# Autodesk Inventor assembly: Gantry
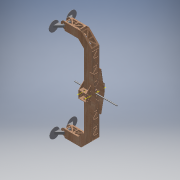
[picture p0: Inventor's stored thumbnail of the model, 180x180]
Saved by Autodesk Inventor 2019 (Build 230136000, 136)
## iProperties
Created: 2019-01-14
Part Number: Gantry
Document SubType Name: Assembly
Designer: nxgam
Author: nxgam
## Documents named in this file (8)
- C:\Users\nxgam\Documents\CAD\Inventor\DiscoDraw\Gantry.iam
- C:\Users\nxgam\Documents\CAD\Inventor\DiscoDraw\Shaft d10.ipt
- C:\Users\nxgam\Documents\CAD\Inventor\DiscoDraw\OctBase.ipt
- C:\Users\nxgam\Documents\CAD\Inventor\DiscoDraw\Leg.iam
- C:\Users\nxgam\Documents\CAD\Inventor\DiscoDraw\OctMiniSupport.ipt
- C:\Users\nxgam\Documents\CAD\Inventor\DiscoDraw\Flange.ipt
- C:\Users\nxgam\Documents\CAD\Inventor\DiscoDraw\SlipRing.ipt
- C:\Users\nxgam\Documents\CAD\Inventor\DiscoDraw\TrusSupport.ipt
## Components (14 placed, 7 different names)
1. Shaft d10:1 — Mate:3, Mate:11, Mate:14
2. OctBase:1 — Mate:1, Flush:3, Flush:4, Mate:2, Mate:3, Flush:14, Flush:15, Mate:13, Flush:16, Flush:19
3. OctBase:2 — Flush:3, Flush:4, Flush:6, Mate:4, Mate:5, Mate:6, Mate:7, Mate:12
4. Leg:1 [sub-assembly] — Flush:1, Flush:2, Mate:1, Flush:6, Flush:7, Angle:1, Flush:16, Mate:18
5. Leg:2 [sub-assembly] — Flush:1, Flush:2, Flush:7, Mate:2, Mate:16, Mate:17
6. OctMiniSupport:1 — Flush:11, Flush:12, Flush:15, Mate:6
7. OctMiniSupport:2 — Flush:10, Flush:11, Flush:12, Mate:7
8. OctMiniSupport:3 — Flush:9, Flush:10, Flush:13, Flush:14, Mate:5
9. OctMiniSupport:4 — Flush:9, Flush:13, Mate:4, Angle:3
10. Flange:1 — Mate:8, Angle:2, Mate:11, Mate:13
11. Flange:2 — Mate:8, Mate:12
12. SlipRing:1 — Mate:14, Angle:3
13. TrusSupport:1 — Mate:16, Flush:19, Flush:20, Flush:21
14. TrusSupport:2 — Mate:17, Flush:20, Flush:21, Mate:18
## Relationships (35: Flush 17, Mate 15, Angle 3)
- Flush:1: Leg:1 ↔ Leg:2
- Flush:2: Leg:1 ↔ Leg:2
- Mate:1: OctBase:1 ↔ Leg:1
- Flush:3: OctBase:1 ↔ OctBase:2
- Flush:4: OctBase:1 ↔ OctBase:2
- Flush:6: OctBase:2 ↔ Leg:1
- Flush:7: Leg:1 ↔ Leg:2
- Angle:1 (0 deg): Leg:1
- Mate:2: OctBase:1 ↔ Leg:2
- Mate:3: Shaft d10:1 ↔ OctBase:1
- Flush:9: OctMiniSupport:3 ↔ OctMiniSupport:4
- Flush:10: OctMiniSupport:2 ↔ OctMiniSupport:3
- Flush:11: OctMiniSupport:1 ↔ OctMiniSupport:2
- Flush:12: OctMiniSupport:1 ↔ OctMiniSupport:2
- Flush:13: OctMiniSupport:3 ↔ OctMiniSupport:4
- Mate:4: OctBase:2 ↔ OctMiniSupport:4
- Flush:14: OctBase:1 ↔ OctMiniSupport:3
- Mate:5: OctBase:2 ↔ OctMiniSupport:3
- Flush:15: OctBase:1 ↔ OctMiniSupport:1
- Mate:6: OctBase:2 ↔ OctMiniSupport:1
- Mate:7: OctBase:2 ↔ OctMiniSupport:2
- Mate:8: Flange:1 ↔ Flange:2
- Angle:2 (0 deg): Flange:1
- Mate:11: Shaft d10:1 ↔ Flange:1
- Mate:12: OctBase:2 ↔ Flange:2
- Mate:13: OctBase:1 ↔ Flange:1
- Mate:14: Shaft d10:1 ↔ SlipRing:1
- Flush:16: OctBase:1 ↔ Leg:1
- Mate:16: Leg:2 ↔ TrusSupport:1
- Flush:19: OctBase:1 ↔ TrusSupport:1
- Mate:17: Leg:2 ↔ TrusSupport:2
- Flush:20: TrusSupport:1 ↔ TrusSupport:2
- Flush:21: TrusSupport:1 ↔ TrusSupport:2
- Mate:18 (-20.32 mm): Leg:1 ↔ TrusSupport:2
- Angle:3 (45 deg): OctMiniSupport:4 ↔ SlipRing:1
